# Autodesk Inventor assembly: Wind Vane Ass
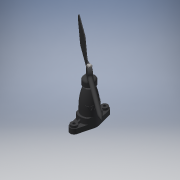
[picture p0: Inventor's stored thumbnail of the model, 180x180]
Saved by Autodesk Inventor 2019 (Build 230136000, 136)
## iProperties
Created: 2020-01-30
Part Number: Wind Vane Ass
Document SubType Name: Assembly
Designer: alb16148
Author: alb16148
## Documents named in this file (11)
- N:\Sandpit\Callum Brooksby\Wind Vane\Wind Vane Ass.iam
- N:\Sandpit\Callum Brooksby\Wind Vane\Base.ipt
- N:\Sandpit\Callum Brooksby\Wind Vane\Lid.ipt
- N:\Sandpit\Callum Brooksby\Wind Vane\Cap.ipt
- N:\Sandpit\Callum Brooksby\Wind Vane\Main Rod.ipt
- N:\Sandpit\Callum Brooksby\anenometer\626-2rs\inafag_626-2rs.iam
- N:\Sandpit\Callum Brooksby\Wind Vane\M6 K-Nut Short.ipt
- N:\Sandpit\Callum Brooksby\Wind Vane\M6 Nut Plain.ipt
- N:\Sandpit\Callum Brooksby\Wind Vane\Tooth Disc.ipt
- N:\Sandpit\Callum Brooksby\Wind Vane\Bottom.ipt
- N:\Sandpit\Callum Brooksby\Wind Vane\Wind Vane.ipt
## Components (15 placed, 10 different names)
1. Base:1 — Insert:1, Insert:5, Mate:2, Mate:3, Mate:4
2. Lid:1 — Insert:1, Insert:2, Insert:4
3. Cap:1 — Insert:2, Insert:12
4. Main Rod:1
5. inafag_626-2rs:1 [sub-assembly] — Insert:4, Insert:6
6. inafag_626-2rs:2 [sub-assembly] — Insert:5, Insert:7, Insert:8
7. M6 K-Nut Short:1 — Insert:7
8. M6 K-Nut Short:2 — Insert:6
9. M6 K-Nut Short:4
10. M6 Nut Plain:1 — Insert:8, Insert:9
11. M6 Nut Plain:2 — Insert:13
12. Tooth Disc:1 — Insert:9, Insert:13
13. M6 K-Nut Short:5 — Insert:12, Insert:14
14. Bottom:1 — Mate:2, Mate:3, Mate:4
15. Wind Vane:1 — Insert:14
## Relationships (14: Insert 11, Mate 3)
- Insert:1: Base:1 ↔ Lid:1
- Insert:2 (1 mm): Lid:1 ↔ Cap:1
- Insert:4: Lid:1 ↔ inafag_626-2rs:1
- Insert:5: Base:1 ↔ inafag_626-2rs:2
- Insert:6: inafag_626-2rs:1 ↔ M6 K-Nut Short:2
- Insert:7: inafag_626-2rs:2 ↔ M6 K-Nut Short:1
- Insert:8: inafag_626-2rs:2 ↔ M6 Nut Plain:1
- Insert:9: M6 Nut Plain:1 ↔ Tooth Disc:1
- Insert:12: Cap:1 ↔ M6 K-Nut Short:5
- Insert:13: M6 Nut Plain:2 ↔ Tooth Disc:1
- Mate:2: Base:1 ↔ Bottom:1
- Mate:3: Base:1 ↔ Bottom:1
- Mate:4: Base:1 ↔ Bottom:1
- Insert:14: M6 K-Nut Short:5 ↔ Wind Vane:1
